# Autodesk Inventor assembly: CoreXY_B
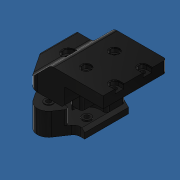
[picture p0: Inventor's stored thumbnail of the model, 180x180]
Saved by Autodesk Inventor 2020 (Build 240168000, 168)
## iProperties
Created: 2021-07-10
Part Number: CoreXY_B
Document SubType Name: Assembly
Designer: ken113
Author: ken113
## Documents named in this file (3)
- D:\Document\Github\Cheap_Belt_Printer\Model\Parts\Print_Parts\Print_Asem\CoreXY_B.iam
- D:\Document\Github\Cheap_Belt_Printer\Model\Parts\Print_Parts\Print_Parts_H_rev2.ipt
- D:\Document\Github\Cheap_Belt_Printer\Model\Parts\Print_Parts\Print_Parts_G_rev2.ipt
## Components (2 placed, 2 different names)
1. Print_Parts_H_rev2:1 — フラッシュ:1, フラッシュ:2, メイト:1
2. Print_Parts_G_rev2:1 — フラッシュ:1, フラッシュ:2, メイト:1
## Relationships (3: Flush 2, Mate 1)
- フラッシュ:1 [Flush]: Print_Parts_H_rev2:1 ↔ Print_Parts_G_rev2:1
- フラッシュ:2 [Flush]: Print_Parts_H_rev2:1 ↔ Print_Parts_G_rev2:1
- メイト:1 [Mate]: Print_Parts_H_rev2:1 ↔ Print_Parts_G_rev2:1
